# Autodesk Inventor assembly: Winch Assembly
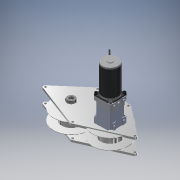
[picture p0: Inventor's stored thumbnail of the model, 180x180]
Saved by Autodesk Inventor 2019.4 (Build 234330000, 330)
## iProperties
Created: 2020-01-24
Part Number: Winch Assembly
Document SubType Name: Assembly
Designer: Mark
Mass: 874.855 g
Surface Area: 1959.09 cm^2
Volume: 436.261 cm^3
Density: 2.00535 g/cm^3
Author: Mark
## Documents named in this file (8)
- C:\Users\Mark\Desktop\7738 Helion Engineering\7738-2020\Ratchet Winch\Winch Assembly.iam
- C:\Users\Mark\Desktop\7738 Helion Engineering\7738-2020\Ratchet Winch\VersaPlanetary_v2_Two_Stage_100_1_with_BAG.ipt
- C:\Users\Mark\Desktop\7738 Helion Engineering\7738-2020\Ratchet Winch\Right Plate.ipt
- C:\Users\Mark\Desktop\7738 Helion Engineering\7738-2020\Ratchet Winch\0_500_Hex_ID_x_1_125_OD_x_0_313_WD_Flanged_Bearing_v2_217-3875.ipt
- C:\Users\Mark\Desktop\7738 Helion Engineering\7738-2020\Elevator MK2\Pulley.ipt
- C:\Users\Mark\Desktop\7738 Helion Engineering\7738-2020\CAD\Gearbox\F6800.ipt
- C:\Users\Mark\Desktop\7738 Helion Engineering\7738-2020\Ratchet Winch\Left Plate.ipt
- C:\Users\Mark\Desktop\7738 Helion Engineering\7738-2020\Elevator MK2\Smol Hex Shaft.ipt
## Components (9 placed, 7 different names)
1. VersaPlanetary_v2_Two_Stage_100_1_with_BAG:1 — Mate:16, Mate:17, Mate:18
2. Right Plate:1 — Mate:4, Mate:5, Mate:9, Mate:10, Mate:11, Flush:3, Mate:14, Flush:4, Flush:5
3. 0_500_Hex_ID_x_1_125_OD_x_0_313_WD_Flanged_Bearing_v2_217-3875:1 — Mate:4, Mate:5, Mate:6
4. Pulley:1 — Mate:6
5. Pulley:2 — Mate:9
6. F6800:1 — Mate:10, Mate:11, Mate:13
7. F6800:2
8. Left Plate:1 — Mate:14, Flush:4, Flush:5, Mate:16, Mate:17, Mate:18
9. Smol Hex Shaft:1 — Mate:13, Flush:3
## Relationships (14: Mate 11, Flush 3)
- Mate:4: Right Plate:1 ↔ 0_500_Hex_ID_x_1_125_OD_x_0_313_WD_Flanged_Bearing_v2_217-3875:1
- Mate:5: Right Plate:1 ↔ 0_500_Hex_ID_x_1_125_OD_x_0_313_WD_Flanged_Bearing_v2_217-3875:1
- Mate:6: 0_500_Hex_ID_x_1_125_OD_x_0_313_WD_Flanged_Bearing_v2_217-3875:1 ↔ Pulley:1
- Mate:9 (1.5 mm): Right Plate:1 ↔ Pulley:2
- Mate:10: Right Plate:1 ↔ F6800:1
- Mate:11: Right Plate:1 ↔ F6800:1
- Mate:13: F6800:1 ↔ Smol Hex Shaft:1
- Flush:3: Right Plate:1 ↔ Smol Hex Shaft:1
- Mate:14 (31 mm): Right Plate:1 ↔ Left Plate:1
- Flush:4: Right Plate:1 ↔ Left Plate:1
- Flush:5: Right Plate:1 ↔ Left Plate:1
- Mate:16: VersaPlanetary_v2_Two_Stage_100_1_with_BAG:1 ↔ Left Plate:1
- Mate:17: VersaPlanetary_v2_Two_Stage_100_1_with_BAG:1 ↔ Left Plate:1
- Mate:18: VersaPlanetary_v2_Two_Stage_100_1_with_BAG:1 ↔ Left Plate:1
